# Autodesk Inventor assembly: cylinder asm
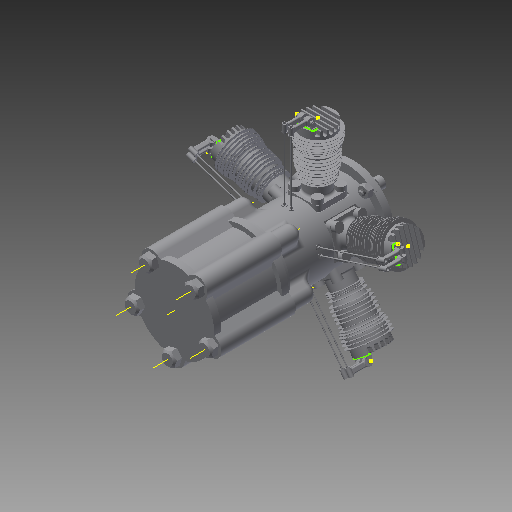
[picture p0: Inventor's stored thumbnail of the model, 512x512]
Saved by Autodesk Inventor 2018 (Build 220112000, 112)
## iProperties
Created: 2021-03-15
Part Number: cylinder asm
Document SubType Name: Assembly
Designer: Jyoti Soni
Author: Jyoti Soni
## Documents named in this file (13)
- C:\Users\Jyoti Soni\Desktop\asm\15032021\cylinder asm.iam
- C:\Users\Jyoti Soni\Desktop\asm\15032021\inner.ipt
- C:\Users\Jyoti Soni\Desktop\asm\15032021\outer.ipt
- C:\Users\Jyoti Soni\Desktop\asm\15032021\lip plate.ipt
- C:\Users\Jyoti Soni\Desktop\asm\15032021\bolt M12x45.ipt
- C:\Users\Jyoti Soni\Desktop\asm\15032021\nut M12.ipt
- C:\Users\Jyoti Soni\Desktop\asm\15032021\bolt M20x200.ipt
- C:\Users\Jyoti Soni\Desktop\asm\15032021\vertical cylinder.ipt
- C:\Users\Jyoti Soni\Desktop\asm\15032021\bolt M10x36.ipt
- C:\Users\Jyoti Soni\Desktop\asm\15032021\pin.ipt
- C:\Users\Jyoti Soni\Desktop\asm\15032021\knuckle.ipt
- C:\Users\Jyoti Soni\Desktop\asm\15032021\lower pin.ipt
- C:\Users\Jyoti Soni\Desktop\asm\15032021\supporting rod.ipt
## Components (88 placed, 12 different names)
1. inner:1 — Mate:1, Mate:2, Mate:3, Mate:8, Insert:3
2. outer:1 — Mate:1, Mate:2, Mate:3, Insert:1, Mate:4, Mate:7, Insert:2, Mate:9, Mate:10, Insert:4
3. lip plate:1 — Insert:1, Mate:4, Mate:5, Mate:6
4. nut M12:1 — Mate:7, Insert:2
5. bolt M12x45:1 — Mate:5, Mate:6
6. nut M12:2
7. bolt M12x45:2
8. nut M12:3
9. bolt M12x45:3
10. nut M12:4
11. bolt M12x45:4
12. nut M12:5
13. bolt M12x45:5
14. bolt M20x200:1 — Mate:8, Insert:3
15. bolt M20x200:2
16. bolt M20x200:3
17. bolt M20x200:4
18. bolt M20x200:5
19. vertical cylinder:1 — Mate:9, Mate:10, Insert:4, Mate:11, Mate:12
20. vertical cylinder:2
21. vertical cylinder:3 — Mate:13, Flush:1, Mate:15, Mate:17, Angle:1, Angle:2
22. vertical cylinder:4
23. vertical cylinder:5
24. lower pin:4 — Mate:24, Mate:25
25. supporting rod:2 — Mate:22, Mate:23, Mate:24, Mate:25
26. supporting rod:1 — Mate:19, Mate:20
27. lower pin:3 — Insert:6, Mate:19, Mate:20
28. lower pin:2 — Mate:18, Mate:21
29. lower pin:1 — Insert:5, Mate:23
30. knuckle:2 — Mate:16, Mate:17, Mate:18, Insert:6, Angle:1, Mate:21
31. knuckle:1 — Mate:14, Mate:15, Insert:5, Angle:2, Mate:22
32. pin:1 — Mate:13, Flush:1, Mate:14, Mate:16
33. lower pin:5
34. supporting rod:3
35. supporting rod:4
36. lower pin:6
37. lower pin:7
38. lower pin:8
39. knuckle:3
40. knuckle:4
41. pin:2
42. lower pin:9
43. supporting rod:5
44. supporting rod:6
45. lower pin:10
46. lower pin:11
47. lower pin:12
48. knuckle:5
49. knuckle:6
50. pin:3
51. lower pin:13
52. supporting rod:7
53. supporting rod:8
54. lower pin:14
55. lower pin:15
56. lower pin:16
57. knuckle:7
58. knuckle:8
59. pin:4
60. lower pin:17
61. supporting rod:9
62. supporting rod:10
63. lower pin:18
64. lower pin:19
65. lower pin:20
66. knuckle:9
67. knuckle:10
68. pin:5
69. bolt M10x36:1 — Mate:11, Mate:12
70. bolt M10x36:2
71. bolt M10x36:3
72. bolt M10x36:4
73. bolt M10x36:5
74. bolt M10x36:6
75. bolt M10x36:7
76. bolt M10x36:8
77. bolt M10x36:9
78. bolt M10x36:10
79. bolt M10x36:11
80. bolt M10x36:12
81. bolt M10x36:13
82. bolt M10x36:14
83. bolt M10x36:15
84. bolt M10x36:16
85. bolt M10x36:17
86. bolt M10x36:18
87. bolt M10x36:19
88. bolt M10x36:20
## Component patterns: (5 elements, first: nut M12:1 + bolt M12x45:1), (5 elements, first: bolt M20x200:1), (5 elements, first: vertical cylinder:1), (5 elements), (5 elements, first: lower pin:4 + supporting rod:2 + supporting rod:1 + lower pin:3 + lower pin:2 + lower pin:1 + knuckle:2 + knuckle:1 + pin:1), (4 elements, first: bolt M10x36:1), Component Pattern 5:2 (4 elements), Component Pattern 5:3 (4 elements), Component Pattern 5:4 (4 elements), Component Pattern 5:5 (4 elements)
## Relationships (34: Mate 25, Insert 6, Angle 2, Flush 1)
- Mate:1: inner:1 ↔ outer:1
- Mate:2: inner:1 ↔ outer:1
- Mate:3: inner:1 ↔ outer:1
- Insert:1: outer:1 ↔ lip plate:1
- Mate:4: outer:1 ↔ lip plate:1
- Mate:5: lip plate:1 ↔ bolt M12x45:1
- Mate:6: lip plate:1 ↔ bolt M12x45:1
- Mate:7: outer:1 ↔ nut M12:1
- Insert:2: outer:1 ↔ nut M12:1
- Mate:8: inner:1 ↔ bolt M20x200:1
- Insert:3: inner:1 ↔ bolt M20x200:1
- Mate:9: outer:1 ↔ vertical cylinder:1
- Mate:10: outer:1 ↔ vertical cylinder:1
- Insert:4: outer:1 ↔ vertical cylinder:1
- Mate:11: vertical cylinder:1 ↔ bolt M10x36:1
- Mate:12: vertical cylinder:1 ↔ bolt M10x36:1
- Mate:13: vertical cylinder:3 ↔ pin:1
- Flush:1 (2 mm): vertical cylinder:3 ↔ pin:1
- Mate:14: knuckle:1 ↔ pin:1
- Mate:15 (2 mm): vertical cylinder:3 ↔ knuckle:1
- Mate:16: knuckle:2 ↔ pin:1
- Mate:17 (2 mm): vertical cylinder:3 ↔ knuckle:2
- Insert:5: lower pin:1 ↔ knuckle:1
- Mate:18: lower pin:2 ↔ knuckle:2
- Insert:6 (140 mm): lower pin:3 ↔ knuckle:2
- Mate:19: supporting rod:1 ↔ lower pin:3
- Mate:20: supporting rod:1 ↔ lower pin:3
- Angle:1 (0 deg): vertical cylinder:3 ↔ knuckle:2
- Angle:2 (0 deg): vertical cylinder:3 ↔ knuckle:1
- Mate:21: lower pin:2 ↔ knuckle:2
- Mate:22: supporting rod:2 ↔ knuckle:1
- Mate:23 (1 mm): supporting rod:2 ↔ lower pin:1
- Mate:24: lower pin:4 ↔ supporting rod:2
- Mate:25: lower pin:4 ↔ supporting rod:2
